# Autodesk Inventor assembly: вт
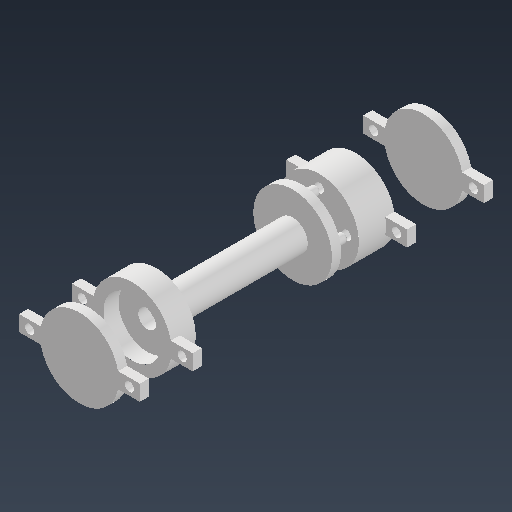
[picture p0: Inventor's stored thumbnail of the model, 512x512]
Saved by Autodesk Inventor 2025 (Build 290162000, 162)
## iProperties
Created: 2025-03-14
Part Number: вт
Document SubType Name: Assembly
Designer: GameHD
Author: GameHD
## Documents named in this file (4)
- C:\Users\GameHD\Desktop\Phantom 16950\вт.iam
- C:\Users\GameHD\Desktop\Phantom 16950\вт3.ipt
- C:\Users\GameHD\Desktop\Phantom 16950\вт1.ipt
- C:\Users\GameHD\Desktop\Phantom 16950\вт2.ipt
## Components (4 placed, 3 different names)
1. вт3:1 — Совмещение:5, Совмещение:6
2. вт1:1 — Совмещение:1, Совмещение:2, Совмещение:5, Совмещение:6
3. вт2:1 — Совмещение:1, Совмещение:2, Совмещение:3, Совмещение:4
4. вт3:2 — Совмещение:3, Совмещение:4
## Relationships (6: Mate 6)
- Совмещение:1 [Mate]: вт1:1 ↔ вт2:1
- Совмещение:2 [Mate]: вт1:1 ↔ вт2:1
- Совмещение:3 [Mate]: вт2:1 ↔ вт3:2
- Совмещение:4 [Mate]: вт2:1 ↔ вт3:2
- Совмещение:5 [Mate]: вт3:1 ↔ вт1:1
- Совмещение:6 [Mate]: вт3:1 ↔ вт1:1
